# Autodesk Inventor assembly: 61545 pinion gear + lock
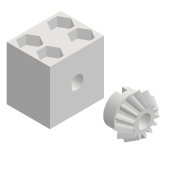
[picture p0: Inventor's stored thumbnail of the model, 180x180]
Saved by Autodesk Inventor 2020 (Build 240168000, 168)
## iProperties
Created: 2019-11-11
Part Number: 61545 pinion gear + lock
Document SubType Name: Assembly
Designer: ball
Author: ball
## Documents named in this file (4)
- C:\FTC\FTC8863CAD\Actobotics\615 parts\61545 pinion gear + lock.iam
- C:\FTC\FTC8863CAD\Actobotics\615 parts\615456_bevel pinion gear.ipt
- C:\FTC\FTC8863CAD\Actobotics\615 parts\Pinion gear lock A.ipt
- C:\FTC\FTC8863CAD\Actobotics\615 parts\615456 bevel gear lock A.ipt
## Components (3 placed, 3 different names)
1. 615456_bevel pinion gear:1 — Flush:1, Mate:1, Angle:1
2. Pinion gear lock A:1 — Flush:1
3. 615456 bevel gear lock A:1 — Mate:1, Angle:1
## Relationships (3: Flush 1, Mate 1, Angle 1)
- Flush:1: 615456_bevel pinion gear:1 ↔ Pinion gear lock A:1
- Mate:1: 615456_bevel pinion gear:1 ↔ 615456 bevel gear lock A:1
- Angle:1 (0 deg): 615456_bevel pinion gear:1 ↔ 615456 bevel gear lock A:1
